# Autodesk Inventor assembly: GP3-100
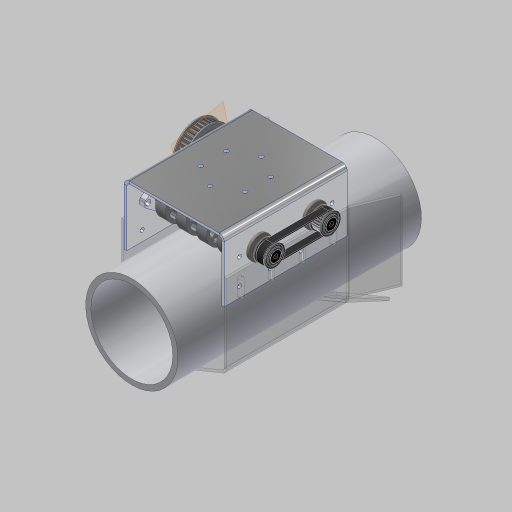
[picture p0: Inventor's stored thumbnail of the model, 512x512]
Saved by Autodesk Inventor 2023.5 (Build 275446000, 446)
## iProperties
Created: 2025-01-14
Part Number: GP3-100
Document SubType Name: Assembly
Designer: brand
Mass: 881.029 g
Surface Area: 5056.84 cm^2
Volume: 1114.3 cm^3
Density: 0.790655 g/cm^3
Author: brand
## Documents named in this file (12)
- C:\Users\slick\OneDrive\Desktop\2025-ReefScape---CAD\Gripper\GP3\GP3-100.iam
- C:\Users\slick\OneDrive\Desktop\2025-ReefScape---CAD\Gripper\GP3\GP3-001.ipt
- C:\Users\slick\OneDrive\Desktop\2025-ReefScape---CAD\Gripper\GP3\GP3-002.ipt
- C:\Users\slick\OneDrive\Desktop\2025-ReefScape---CAD\Field Items\Game Pieces\GE-25500.ipt
- C:\Users\slick\OneDrive\Desktop\2025-ReefScape---CAD\COMMON PARTS\BEARINGS\0_500_Hex_ID_x_1_125_OD_x_0_313_WD_Flanged_Bearing_v2_217-3875.ipt
- C:\Users\slick\OneDrive\Desktop\2025-ReefScape---CAD\COMMON PARTS\WHEELS\1_625_OD_Straight_Flex_Wheel_217-6350.ipt
- C:\Users\slick\OneDrive\Desktop\2025-ReefScape---CAD\COMMON PARTS\PULLEYS\gt2\24t_x_9mm_Wide_Double_Flange_Aluminum_Pulley_GT2_3mm_1_2_Hex_Bore_217-5875.ipt
- C:\Users\slick\OneDrive\Desktop\2025-ReefScape---CAD\Gripper\GP3\GP3-003.ipt
- C:\Users\slick\OneDrive\Desktop\2025-ReefScape---CAD\Gripper\GP3\GP3-004.ipt
- C:\Users\slick\OneDrive\Desktop\2025-ReefScape---CAD\Gripper\GP3\GP3-005.ipt
- C:\Users\slick\OneDrive\Desktop\2025-ReefScape---CAD\COMMON PARTS\PULLEYS\htd\36t_x_9mm_Wide_Double_Flange_Aluminum_Pulley_HTD_5mm_1_2_Hex_Bore_217-3231.ipt
- C:\Users\slick\OneDrive\Desktop\2025-ReefScape---CAD\COMMON PARTS\BEARINGS\Bearing Retainer\Retainer.ipt
## Components (25 placed, 11 different names)
1. GP3-001:1 — Flush:1, Insert:1, Insert:2, Insert:3, Insert:4, Mate:16, Flush:9, Insert:5, Insert:6, Insert:7, Insert:8, Insert:9, Insert:10, Insert:11, Insert:12
2. GP3-002:1 — Flush:1, Mate:16, Tangent:2, Tangent:3, Flush:9
3. GE-25500:1 — Tangent:2, Tangent:3
4. 0_500_Hex_ID_x_1_125_OD_x_0_313_WD_Flanged_Bearing_v2_217-3875:1 — Insert:1, Mate:17
5. 0_500_Hex_ID_x_1_125_OD_x_0_313_WD_Flanged_Bearing_v2_217-3875:2 — Insert:2, Mate:5, Mate:13, Mate:18
6. 0_500_Hex_ID_x_1_125_OD_x_0_313_WD_Flanged_Bearing_v2_217-3875:3 — Insert:3, Mate:3
7. 0_500_Hex_ID_x_1_125_OD_x_0_313_WD_Flanged_Bearing_v2_217-3875:4 — Insert:4, Mate:2, Mate:15
8. 24t_x_9mm_Wide_Double_Flange_Aluminum_Pulley_GT2_3mm_1_2_Hex_Bore_217-5875:1 — Mate:6, Flush:2, Flush:5, Flush:6, Mate:13
9. 24t_x_9mm_Wide_Double_Flange_Aluminum_Pulley_GT2_3mm_1_2_Hex_Bore_217-5875:2 — Flush:2, Tangent:1, Flush:8
10. GP3-005:1 — Mate:14, Flush:8
11. GP3-003:2 — Mate:5, Mate:6, Mate:7, Mate:8, Mate:12, Flush:6
12. GP3-004:1 — Mate:12, Tangent:1, Flush:5
13. 36t_x_9mm_Wide_Double_Flange_Aluminum_Pulley_HTD_5mm_1_2_Hex_Bore_217-3231:1 — Mate:14, Mate:15
14. Retainer:1 — Insert:5, Insert:6
15. Retainer:2 — Insert:7, Insert:8
16. Retainer:3 — Insert:9, Insert:10
17. Retainer:4 — Insert:11, Insert:12
18. 1_625_OD_Straight_Flex_Wheel_217-6350:3 — Mate:7, Flush:3, Mate:18
19. 1_625_OD_Straight_Flex_Wheel_217-6350:2 — Mate:3, Flush:3
20. 1_625_OD_Straight_Flex_Wheel_217-6350:5
21. 1_625_OD_Straight_Flex_Wheel_217-6350:6
22. 1_625_OD_Straight_Flex_Wheel_217-6350:4 — Mate:8, Flush:4, Mate:17
23. 1_625_OD_Straight_Flex_Wheel_217-6350:1 — Mate:2, Flush:4
24. 1_625_OD_Straight_Flex_Wheel_217-6350:7
25. 1_625_OD_Straight_Flex_Wheel_217-6350:8
## Component patterns: (2 elements, first: 1_625_OD_Straight_Flex_Wheel_217-6350:3 + 1_625_OD_Straight_Flex_Wheel_217-6350:2), (2 elements, first: 1_625_OD_Straight_Flex_Wheel_217-6350:4 + 1_625_OD_Straight_Flex_Wheel_217-6350:1)
## Relationships (38: Mate 15, Insert 12, Flush 8, Tangent 3)
- Flush:1: GP3-001:1 ↔ GP3-002:1
- Insert:1: GP3-001:1 ↔ 0_500_Hex_ID_x_1_125_OD_x_0_313_WD_Flanged_Bearing_v2_217-3875:1
- Insert:2: GP3-001:1 ↔ 0_500_Hex_ID_x_1_125_OD_x_0_313_WD_Flanged_Bearing_v2_217-3875:2
- Insert:3: GP3-001:1 ↔ 0_500_Hex_ID_x_1_125_OD_x_0_313_WD_Flanged_Bearing_v2_217-3875:3
- Insert:4: GP3-001:1 ↔ 0_500_Hex_ID_x_1_125_OD_x_0_313_WD_Flanged_Bearing_v2_217-3875:4
- Mate:2: 0_500_Hex_ID_x_1_125_OD_x_0_313_WD_Flanged_Bearing_v2_217-3875:4 ↔ 1_625_OD_Straight_Flex_Wheel_217-6350:1
- Mate:3: 0_500_Hex_ID_x_1_125_OD_x_0_313_WD_Flanged_Bearing_v2_217-3875:3 ↔ 1_625_OD_Straight_Flex_Wheel_217-6350:2
- Mate:5: 0_500_Hex_ID_x_1_125_OD_x_0_313_WD_Flanged_Bearing_v2_217-3875:2 ↔ GP3-003:2
- Mate:6: 24t_x_9mm_Wide_Double_Flange_Aluminum_Pulley_GT2_3mm_1_2_Hex_Bore_217-5875:1 ↔ GP3-003:2
- Mate:7: GP3-003:2 ↔ 1_625_OD_Straight_Flex_Wheel_217-6350:3
- Mate:8: GP3-003:2 ↔ 1_625_OD_Straight_Flex_Wheel_217-6350:4
- [Mate]: 0_500_Hex_ID_x_1_125_OD_x_0_313_WD_Flanged_Bearing_v2_217-3875:3 ↔ GP3-005:1
- [Mate]: 24t_x_9mm_Wide_Double_Flange_Aluminum_Pulley_GT2_3mm_1_2_Hex_Bore_217-5875:2 ↔ GP3-005:1
- Flush:2: 24t_x_9mm_Wide_Double_Flange_Aluminum_Pulley_GT2_3mm_1_2_Hex_Bore_217-5875:1 ↔ 24t_x_9mm_Wide_Double_Flange_Aluminum_Pulley_GT2_3mm_1_2_Hex_Bore_217-5875:2
- Flush:3: 1_625_OD_Straight_Flex_Wheel_217-6350:3 ↔ 1_625_OD_Straight_Flex_Wheel_217-6350:2
- Flush:4: 1_625_OD_Straight_Flex_Wheel_217-6350:4 ↔ 1_625_OD_Straight_Flex_Wheel_217-6350:1
- Mate:12: GP3-003:2 ↔ GP3-004:1
- Tangent:1: 24t_x_9mm_Wide_Double_Flange_Aluminum_Pulley_GT2_3mm_1_2_Hex_Bore_217-5875:2 ↔ GP3-004:1
- Flush:5: 24t_x_9mm_Wide_Double_Flange_Aluminum_Pulley_GT2_3mm_1_2_Hex_Bore_217-5875:1 ↔ GP3-004:1
- Flush:6: 24t_x_9mm_Wide_Double_Flange_Aluminum_Pulley_GT2_3mm_1_2_Hex_Bore_217-5875:1 ↔ GP3-003:2
- Mate:13 (3.175 mm): 0_500_Hex_ID_x_1_125_OD_x_0_313_WD_Flanged_Bearing_v2_217-3875:2 ↔ 24t_x_9mm_Wide_Double_Flange_Aluminum_Pulley_GT2_3mm_1_2_Hex_Bore_217-5875:1
- Mate:14: GP3-005:1 ↔ 36t_x_9mm_Wide_Double_Flange_Aluminum_Pulley_HTD_5mm_1_2_Hex_Bore_217-3231:1
- Flush:8: 24t_x_9mm_Wide_Double_Flange_Aluminum_Pulley_GT2_3mm_1_2_Hex_Bore_217-5875:2 ↔ GP3-005:1
- Mate:15 (3.175 mm): 0_500_Hex_ID_x_1_125_OD_x_0_313_WD_Flanged_Bearing_v2_217-3875:4 ↔ 36t_x_9mm_Wide_Double_Flange_Aluminum_Pulley_HTD_5mm_1_2_Hex_Bore_217-3231:1
- Mate:16: GP3-001:1 ↔ GP3-002:1
- Tangent:2: GP3-002:1 ↔ GE-25500:1
- Tangent:3: GP3-002:1 ↔ GE-25500:1
- Mate:17 (38.1 mm): 0_500_Hex_ID_x_1_125_OD_x_0_313_WD_Flanged_Bearing_v2_217-3875:1 ↔ 1_625_OD_Straight_Flex_Wheel_217-6350:4
- Mate:18 (38.1 mm): 0_500_Hex_ID_x_1_125_OD_x_0_313_WD_Flanged_Bearing_v2_217-3875:2 ↔ 1_625_OD_Straight_Flex_Wheel_217-6350:3
- Flush:9: GP3-001:1 ↔ GP3-002:1
- Insert:5: GP3-001:1 ↔ Retainer:1
- Insert:6: GP3-001:1 ↔ Retainer:1
- Insert:7: GP3-001:1 ↔ Retainer:2
- Insert:8: GP3-001:1 ↔ Retainer:2
- Insert:9: GP3-001:1 ↔ Retainer:3
- Insert:10: GP3-001:1 ↔ Retainer:3
- Insert:11: GP3-001:1 ↔ Retainer:4
- Insert:12: GP3-001:1 ↔ Retainer:4
